# Autodesk Inventor assembly: plunger assembly
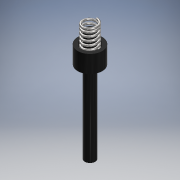
[picture p0: Inventor's stored thumbnail of the model, 180x180]
Saved by Autodesk Inventor 2022 (Build 260153000, 153)
## iProperties
Created: 2022-02-18
Part Number: plunger assembly
Document SubType Name: Assembly
Designer: Bowen
Author: Bowen
## Documents named in this file (3)
- C:\$WorkingFolder\Engineering Data\MemeSat\Switches\plunger assembly.iam
- C:\$WorkingFolder\Engineering Data\MemeSat\Switches\plunger extension.ipt
- C:\$WorkingFolder\Engineering Data\MemeSat\Switches\9657K236_Compression Spring.ipt
## Components (2 placed, 2 different names)
1. plunger extension:1 — Mate:1, Mate:2, Flush:1, Flush:2, Flush:3, Mate:3
2. 9657K236_Compression Spring:1 — Mate:1, Mate:2, Mate:3
## Relationships (6: Mate 3, Flush 3)
- Mate:1: plunger extension:1 ↔ 9657K236_Compression Spring:1
- Mate:2: plunger extension:1 ↔ 9657K236_Compression Spring:1
- Flush:1: plunger extension:1
- Flush:2: plunger extension:1
- Flush:3: plunger extension:1
- Mate:3 (0.1524 mm): plunger extension:1 ↔ 9657K236_Compression Spring:1
